# Autodesk Inventor assembly: Assembly4
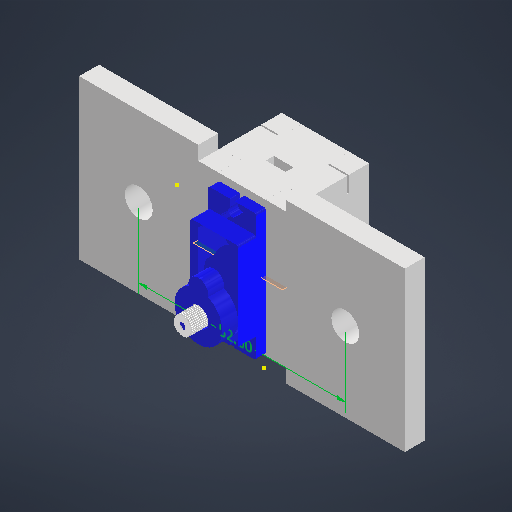
[picture p0: Inventor's stored thumbnail of the model, 512x512]
Saved by Autodesk Inventor 2026.2 (Build 302298000, 298)
## iProperties
Created: 2026-04-17
Part Number: Assembly4
Document SubType Name: Assembly
Designer: danda
Author: danda
## Documents named in this file (5)
- C:\Users\danda\BOM-project\Project\CAD\sorting\Towerpro Micro Servo 9g\Towerpro Micro Servo 9g\Assembly4.iam
- C:\Users\danda\BOM-project\Project\CAD\sorting\Towerpro Micro Servo 9g\Part7.ipt
- C:\Users\danda\BOM-project\Project\CAD\sorting\Towerpro Micro Servo 9g\Part6.ipt
- C:\Users\danda\BOM-project\Project\CAD\sorting\Towerpro Micro Servo 9g\Towerpro Micro Servo 9g\Towerpro Micro Servo 9g_MIR.ipt
- C:\Users\danda\BOM-project\Project\CAD\sorting\Towerpro Micro Servo 9g\Towerpro Micro Servo 9g\Part8.ipt
## Components (7 placed, 4 different names)
1. Part7:1 — Flush:5, Flush:6, Flush:7, Mate:4, Mate:5, Flush:8, Flush:9, Flush:10
2. Part6:1 — Flush:8, Flush:9, Flush:10, Flush:11, Flush:12, Flush:13, Mate:10, Mate:11, Mate:12, Mate:13
3. Part7:2 — Flush:11, Mate:9, Flush:12, Flush:13
4. Part6:2 — Flush:5, Flush:6, Flush:7, Mate:6, Mate:7, Mate:8, Mate:9
5. Towerpro Micro Servo 9g_MIR:1 — Mate:4, Mate:5, Mate:10
6. Part8:1 — Mate:6, Mate:7, Mate:8
7. Part8:2 — Mate:11, Mate:12, Mate:13
## Relationships (19: Mate 10, Flush 9)
- Flush:5: Part7:1 ↔ Part6:2
- Flush:6: Part7:1 ↔ Part6:2
- Flush:7: Part7:1 ↔ Part6:2
- Mate:4: Part7:1 ↔ Towerpro Micro Servo 9g_MIR:1
- Mate:5: Part7:1 ↔ Towerpro Micro Servo 9g_MIR:1
- Mate:6: Part6:2 ↔ Part8:1
- Mate:7: Part6:2 ↔ Part8:1
- Mate:8: Part6:2 ↔ Part8:1
- Flush:8: Part7:1 ↔ Part6:1
- Flush:9: Part7:1 ↔ Part6:1
- Flush:10: Part7:1 ↔ Part6:1
- Flush:11: Part6:1 ↔ Part7:2
- Mate:9: Part7:2 ↔ Part6:2
- Flush:12: Part6:1 ↔ Part7:2
- Flush:13: Part6:1 ↔ Part7:2
- Mate:10: Part6:1 ↔ Towerpro Micro Servo 9g_MIR:1
- Mate:11: Part6:1 ↔ Part8:2
- Mate:12: Part6:1 ↔ Part8:2
- Mate:13: Part6:1 ↔ Part8:2
